# Autodesk Inventor assembly: Torso
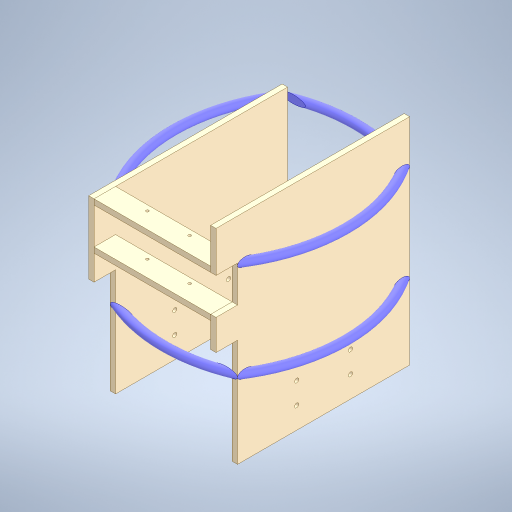
[picture p0: Inventor's stored thumbnail of the model, 512x512]
Saved by Autodesk Inventor 2024 (Build 280153000, 153)
## iProperties
Created: 2024-03-21
Part Number: Torso
Document SubType Name: Assembly
Designer: Liz
Author: Liz
## Documents named in this file (6)
- C:\Users\anyangoe\Desktop\WholeRobot\Torso.iam
- C:\Users\anyangoe\Desktop\WholeRobot\Wood-6.ipt
- C:\Users\anyangoe\Desktop\WholeRobot\Wood-7.ipt
- C:\Users\anyangoe\Desktop\WholeRobot\Wood-8.ipt
- C:\Users\anyangoe\Desktop\WholeRobot\Hula Hoop-1.ipt
- C:\Users\anyangoe\Desktop\WholeRobot\Hula Hoop-2.ipt
## Components (11 placed, 5 different names)
1. Wood-6:1 — Flush:3, Flush:4, Mate:1, Mate:3, Mate:4, Mate:5, Flush:7, Mate:7, Mate:8, Mate:9, Mate:12, Flush:9
2. Wood-7:1 — Flush:3, Flush:4, Mate:1, Mate:2, Flush:5, Flush:6, Mate:14, Mate:15, Mate:19, Mate:21
3. Wood-8:1 — Mate:2, Flush:5, Flush:6, Mate:20
4. Hula Hoop-1:1 — Mate:5, Flush:7, Mate:6, Mate:18, Flush:10
5. Hula Hoop-1:2 — Mate:3, Mate:4, Mate:6, Mate:7, Mate:11, Mate:17
6. Hula Hoop-2:1 — Mate:9, Mate:10, Flush:8, Mate:22
7. Hula Hoop-2:2 — Mate:8, Mate:10, Mate:11, Mate:12, Flush:8, Mate:16
8. Hula Hoop-1:3 — Mate:14, Mate:18
9. Hula Hoop-1:4 — Mate:15, Mate:16, Mate:17
10. Wood-8:2 — Mate:19, Flush:9, Mate:20
11. Hula Hoop-2:3 — Mate:21, Flush:10, Mate:22
## Relationships (30: Mate 22, Flush 8)
- Flush:3: Wood-6:1 ↔ Wood-7:1
- Flush:4: Wood-6:1 ↔ Wood-7:1
- Mate:1 (275.4 mm): Wood-6:1 ↔ Wood-7:1
- Mate:2: Wood-7:1 ↔ Wood-8:1
- Flush:5: Wood-7:1 ↔ Wood-8:1
- Flush:6: Wood-7:1 ↔ Wood-8:1
- Mate:3: Wood-6:1 ↔ Hula Hoop-1:2
- Mate:4: Wood-6:1 ↔ Hula Hoop-1:2
- Mate:5: Wood-6:1 ↔ Hula Hoop-1:1
- Flush:7: Wood-6:1 ↔ Hula Hoop-1:1
- Mate:6 (-228.6 mm): Hula Hoop-1:1 ↔ Hula Hoop-1:2
- Mate:7 (-76.2 mm): Wood-6:1 ↔ Hula Hoop-1:2
- Mate:8: Wood-6:1 ↔ Hula Hoop-2:2
- Mate:9: Wood-6:1 ↔ Hula Hoop-2:1
- Mate:10: Hula Hoop-2:1 ↔ Hula Hoop-2:2
- Mate:11: Hula Hoop-1:2 ↔ Hula Hoop-2:2
- Mate:12 (-150.4 mm): Wood-6:1 ↔ Hula Hoop-2:2
- Flush:8: Hula Hoop-2:1 ↔ Hula Hoop-2:2
- [Mate] (-228.6 mm): Hula Hoop-1:3 ↔ Hula Hoop-1:4
- Mate:14: Wood-7:1 ↔ Hula Hoop-1:3
- Mate:15: Wood-7:1 ↔ Hula Hoop-1:4
- Mate:16: Hula Hoop-2:2 ↔ Hula Hoop-1:4
- Mate:17: Hula Hoop-1:2 ↔ Hula Hoop-1:4
- Mate:18: Hula Hoop-1:1 ↔ Hula Hoop-1:3
- Mate:19: Wood-7:1 ↔ Wood-8:2
- Flush:9: Wood-6:1 ↔ Wood-8:2
- Mate:20: Wood-8:1 ↔ Wood-8:2
- Mate:21: Wood-7:1 ↔ Hula Hoop-2:3
- Flush:10: Hula Hoop-1:1 ↔ Hula Hoop-2:3
- Mate:22: Hula Hoop-2:1 ↔ Hula Hoop-2:3
## Named parameters: d27_d19 = -228.6 mm
